# Autodesk Inventor assembly: 64 to 12 Single Stage Gearbox
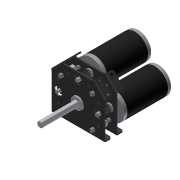
[picture p0: Inventor's stored thumbnail of the model, 180x180]
Saved by Autodesk Inventor 2013 (Build 170138000, 138)
## iProperties
Created: 2013-01-06
Part Number: 64 to 12 Single Stage Gearbox
Document SubType Name: Assembly
Designer: Nemo
Author: Nemo
## Documents named in this file (10)
- H:\Nemo\Documents\Robotics\COTS Parts\Gearboxes\VexPro 64 Single Stage Gearbox.iam
- H:\Nemo\Documents\Robotics\COTS Parts\Gearboxes\Components\VexPro Single Stage Components\64 single stage gearbox plate.ipt
- H:\Nemo\Documents\Robotics\COTS Parts\Bearings - VexPro\Flanged Bearing - 0.5in Round ID x 1.125in OD.ipt
- H:\Nemo\Documents\Robotics\COTS Parts\Bearings - VexPro\Flanged Bearing - 0.5in Hex ID x 1.125in OD.ipt
- H:\Nemo\Documents\Robotics\COTS Parts\Gearboxes\Components\VexPro Single Stage Components\Single stage gearbox output shaft.ipt
- H:\Nemo\Documents\Robotics\COTS Parts\Gears - VexPro\Gear 20dp 500hex 64T Vex.ipt
- H:\Nemo\Documents\Robotics\COTS Parts\Fasteners\500 Hex Coupler.ipt
- H:\Nemo\Documents\Robotics\COTS Parts\Fasteners\Hex Standoff 14-20 x1000.ipt
- H:\Nemo\Documents\Robotics\COTS Parts\Fasteners\14-20 SHCS x500.ipt
- H:\Nemo\Documents\Robotics\COTS Parts\Gearboxes\Components\VexPro Single Stage Components\CIM for Single Stage Vex Box.iam
## Components (22 placed, 9 different names)
1. 64 single stage gearbox plate:1 — Mate:1, Mate:2, Mate:3, Insert:1, Insert:12, Insert:13, Insert:14, Insert:15, Insert:19, Mate:9, Insert:20, Mate:10, Insert:21, Mate:11
2. 64 single stage gearbox plate:2 — Mate:1, Mate:2, Mate:3, Insert:2, Insert:4, Insert:5, Insert:6, Insert:7, Insert:8, Insert:9, Insert:10, Insert:11
3. Flanged Bearing - 0.5in Round ID x 1.125in OD:1 — Insert:1, Insert:3
4. Flanged Bearing - 0.5in Hex ID x 1.125in OD:1 — Insert:2, Angle:1, Mate:5
5. Single stage gearbox output shaft:1 — Insert:3, Angle:1, Mate:4, Angle:2, Mate:6, Angle:3
6. Gear 20dp 500hex 64T Vex:1 — Mate:4, Angle:2, Mate:5, Mate:7
7. 500 Hex Coupler:1 — Mate:6, Angle:3, Mate:7
8. Hex Standoff 14-20 x1000:1 — Insert:4
9. Hex Standoff 14-20 x1000:2 — Insert:5
10. Hex Standoff 14-20 x1000:3 — Insert:7
11. Hex Standoff 14-20 x1000:4 — Insert:6
12. 14-20 SHCS x500:1 — Insert:13
13. 14-20 SHCS x500:2 — Insert:14
14. 14-20 SHCS x500:3 — Insert:10
15. 14-20 SHCS x500:4 — Insert:8
16. 14-20 SHCS x500:5 — Insert:9
17. 14-20 SHCS x500:6 — Insert:15
18. 14-20 SHCS x500:7 — Insert:12
19. 14-20 SHCS x500:8 — Insert:11
20. CIM for Single Stage Vex Box:2 [sub-assembly] — Insert:19, Mate:9
21. CIM for Single Stage Vex Box:3 [sub-assembly] — Insert:20, Mate:10
22. CIM for Single Stage Vex Box:4 [sub-assembly] — Insert:21, Mate:11
## Relationships (31: Insert 18, Mate 10, Angle 3)
- Mate:1: 64 single stage gearbox plate:1 ↔ 64 single stage gearbox plate:2
- Mate:2: 64 single stage gearbox plate:1 ↔ 64 single stage gearbox plate:2
- Mate:3 (25.4 mm): 64 single stage gearbox plate:1 ↔ 64 single stage gearbox plate:2
- Insert:1: 64 single stage gearbox plate:1 ↔ Flanged Bearing - 0.5in Round ID x 1.125in OD:1
- Insert:2: 64 single stage gearbox plate:2 ↔ Flanged Bearing - 0.5in Hex ID x 1.125in OD:1
- Insert:3: Flanged Bearing - 0.5in Round ID x 1.125in OD:1 ↔ Single stage gearbox output shaft:1
- Angle:1 (0 deg): Flanged Bearing - 0.5in Hex ID x 1.125in OD:1 ↔ Single stage gearbox output shaft:1
- Mate:4: Single stage gearbox output shaft:1 ↔ Gear 20dp 500hex 64T Vex:1
- Angle:2 (0 deg): Single stage gearbox output shaft:1 ↔ Gear 20dp 500hex 64T Vex:1
- Mate:5: Flanged Bearing - 0.5in Hex ID x 1.125in OD:1 ↔ Gear 20dp 500hex 64T Vex:1
- Mate:6: Single stage gearbox output shaft:1 ↔ 500 Hex Coupler:1
- Angle:3 (0 deg): Single stage gearbox output shaft:1 ↔ 500 Hex Coupler:1
- Mate:7: Gear 20dp 500hex 64T Vex:1 ↔ 500 Hex Coupler:1
- Insert:4: 64 single stage gearbox plate:2 ↔ Hex Standoff 14-20 x1000:1
- Insert:5: 64 single stage gearbox plate:2 ↔ Hex Standoff 14-20 x1000:2
- Insert:6: 64 single stage gearbox plate:2 ↔ Hex Standoff 14-20 x1000:4
- Insert:7: 64 single stage gearbox plate:2 ↔ Hex Standoff 14-20 x1000:3
- Insert:8: 64 single stage gearbox plate:2 ↔ 14-20 SHCS x500:4
- Insert:9: 64 single stage gearbox plate:2 ↔ 14-20 SHCS x500:5
- Insert:10: 64 single stage gearbox plate:2 ↔ 14-20 SHCS x500:3
- Insert:11: 64 single stage gearbox plate:2 ↔ 14-20 SHCS x500:8
- Insert:12: 64 single stage gearbox plate:1 ↔ 14-20 SHCS x500:7
- Insert:13: 64 single stage gearbox plate:1 ↔ 14-20 SHCS x500:1
- Insert:14: 64 single stage gearbox plate:1 ↔ 14-20 SHCS x500:2
- Insert:15: 64 single stage gearbox plate:1 ↔ 14-20 SHCS x500:6
- Insert:19: 64 single stage gearbox plate:1 ↔ CIM for Single Stage Vex Box:2
- Mate:9: 64 single stage gearbox plate:1 ↔ CIM for Single Stage Vex Box:2
- Insert:20: 64 single stage gearbox plate:1 ↔ CIM for Single Stage Vex Box:3
- Mate:10: 64 single stage gearbox plate:1 ↔ CIM for Single Stage Vex Box:3
- Insert:21: 64 single stage gearbox plate:1 ↔ CIM for Single Stage Vex Box:4
- Mate:11: 64 single stage gearbox plate:1 ↔ CIM for Single Stage Vex Box:4
